# Autodesk Inventor assembly: Seilrolle
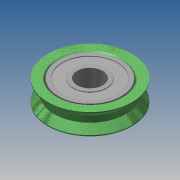
[picture p0: Inventor's stored thumbnail of the model, 180x180]
Saved by Autodesk Inventor 2015 SP1 (Build 190203100, 203)
## iProperties
Created: 2015-02-20
Part Number: Seilrolle
Document SubType Name: Assembly
Designer: Marc
Author: Marc
## Documents named in this file (3)
- E:\Modellflieger\3D Drucker\MotediusQR 500mm\Z-Achse\Seilrolle.iam
- E:\Modellflieger\3D Drucker\MotediusQR 500mm\Z-Achse\Seilrolle.ipt
- E:\Modellflieger\3D Drucker\Eigene Teile\Kugellager_6x15x5_696ZZ.ipt
## Components (2 placed, 2 different names)
1. Seilrolle:1 — Einfügen:1
2. Kugellager_6x15x5_696ZZ:1 — Einfügen:1
## Relationships (1: Insert 1)
- Einfügen:1 [Insert]: Seilrolle:1 ↔ Kugellager_6x15x5_696ZZ:1
